# Autodesk Inventor assembly: BielaMestraEquipada
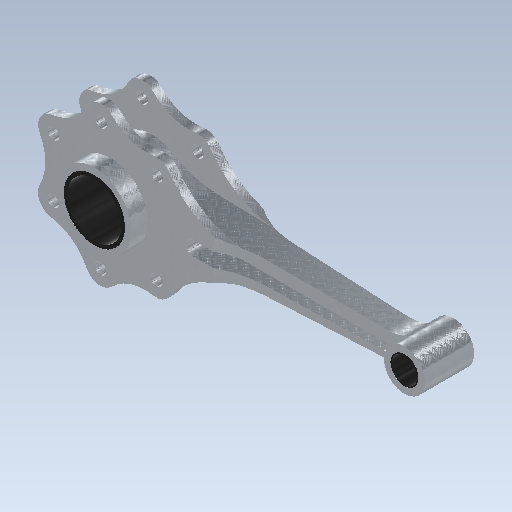
[picture p0: Inventor's stored thumbnail of the model, 512x512]
Saved by Autodesk Inventor 2021 (Build 250183000, 183)
## iProperties
Category: 10
Company: UFABC
Created: 2021-07-26
Document SubType Name: Assembly
Designer: Giovanni
Checked By: Prof. Luis
User Status: 1:5
Description: 01
Author: Giovanni Rodrigues Dias
Keywords: 3
Revision Number: 01
## Documents named in this file (4)
- C:\Users\irineu\Documents\Inventor\MotorRadial7\BielaMestraEquipada.iam
- C:\Users\irineu\Documents\Inventor\MotorRadial7\Bucha Biela Mestra.ipt
- C:\Users\irineu\Documents\Inventor\MotorRadial7\Bucha Superior.ipt
- C:\Users\irineu\Documents\Inventor\MotorRadial7\Biela Mestra.ipt
## Components (3 placed, 3 different names)
1. Biela Mestra:1 — Inserir:1, Inserir:2
2. Bucha Biela Mestra:1 — Inserir:1
3. Bucha Superior:1 — Inserir:2
## Relationships (2: Insert 2)
- Inserir:1: Biela Mestra:1 ↔ Bucha Biela Mestra:1
- Inserir:2: Biela Mestra:1 ↔ Bucha Superior:1
